# Autodesk Inventor assembly: Inner Assembly
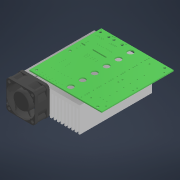
[picture p0: Inventor's stored thumbnail of the model, 180x180]
Saved by Autodesk Inventor 2022 (Build 260153000, 153)
## iProperties
Created: 2023-06-09
Part Number: Inner Assembly
Document SubType Name: Assembly
Designer: voids
Author: voids
## Documents named in this file (4)
- C:\Users\voids\Desktop\Projects\CLASS C PROJECTS\CNC Controller\HV servo drive v1\Inner Assembly.iam
- C:\Users\voids\Desktop\Projects\CLASS C PROJECTS\CNC Controller\HV servo drive v1\heatsink.ipt
- C:\Users\voids\Desktop\Projects\CLASS C PROJECTS\CNC Controller\HV servo drive v1\PCB v1.iam
- C:\Users\voids\Desktop\Projects\CLASS C PROJECTS\CNC Controller\HV servo drive v1\SanAce_9GA_40x20_RBD.ipt
## Components (3 placed, 3 different names)
1. heatsink:1 — Mate:1, Mate:2, Mate:3
2. PCB v1:1 [sub-assembly] — Mate:1, Mate:2, Mate:3
3. SanAce_9GA_40x20_RBD:1
## Relationships (3: Mate 3)
- Mate:1 (6 mm): heatsink:1 ↔ PCB v1:1
- Mate:2: heatsink:1 ↔ PCB v1:1
- Mate:3: heatsink:1 ↔ PCB v1:1
